# Autodesk Inventor assembly: Frame 1647030135921
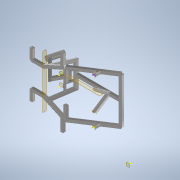
[picture p0: Inventor's stored thumbnail of the model, 180x180]
Saved by Autodesk Inventor 2022.2 (Build 262287000, 287)
## iProperties
_FrameDoc: Frame Assembly
_Version: 25.0.0
Created: 2022-03-11
Part Number: Frame 1647030135921
Document SubType Name: Assembly
Designer: foriw
Mass: 3942.11 g
Surface Area: 4958.76 cm^2
Volume: 504.942 cm^3
Density: 7.80705 g/cm^3
Author: foriw
## Documents named in this file (29)
- C:\Users\foriw\OneDrive\Dokumenter\Inventor\BeerCart - Github - Mekatronik\BeerCart-CAD-Inventor\Workspaces\Workspace\beercart assembly - mekatronik\Frame\Frame 1647030135921.iam
- C:\Users\foriw\OneDrive\Dokumenter\Inventor\BeerCart - Github - Mekatronik\BeerCart-CAD-Inventor\Workspaces\Workspace\beercart assembly - mekatronik\Frame\Skeleton 1647030135922.ipt
- C:\Users\foriw\OneDrive\Dokumenter\Inventor\BeerCart - Github - Mekatronik\BeerCart-CAD-Inventor\Workspaces\Workspace\beercart assembly - mekatronik\Frame\ISO 12633-2 20x20x2 1647030137505.ipt
- C:\Users\foriw\OneDrive\Dokumenter\Inventor\BeerCart - Github - Mekatronik\BeerCart-CAD-Inventor\Workspaces\Workspace\beercart assembly - mekatronik\Frame\ISO 12633-2 20x20x2 1647030138110.ipt
- C:\Users\foriw\OneDrive\Dokumenter\Inventor\BeerCart - Github - Mekatronik\BeerCart-CAD-Inventor\Workspaces\Workspace\beercart assembly - mekatronik\Frame\ISO 12633-2 20x20x2 1647030138225.ipt
- C:\Users\foriw\OneDrive\Dokumenter\Inventor\BeerCart - Github - Mekatronik\BeerCart-CAD-Inventor\Workspaces\Workspace\beercart assembly - mekatronik\Frame\ISO 12633-2 20x20x2 1647030639616.ipt
- C:\Users\foriw\OneDrive\Dokumenter\Inventor\BeerCart - Github - Mekatronik\BeerCart-CAD-Inventor\Workspaces\Workspace\beercart assembly - mekatronik\Frame\ISO 12633-2 20x20x2 1647030639707.ipt
- C:\Users\foriw\OneDrive\Dokumenter\Inventor\BeerCart - Github - Mekatronik\BeerCart-CAD-Inventor\Workspaces\Workspace\beercart assembly - mekatronik\Frame\ISO 1035_2 10x 10 1647602096505.ipt
- C:\Users\foriw\OneDrive\Dokumenter\Inventor\BeerCart - Github - Mekatronik\BeerCart-CAD-Inventor\Workspaces\Workspace\beercart assembly - mekatronik\Frame\ISO 1035_2 10x 10 1647602096566.ipt
- C:\Users\foriw\OneDrive\Dokumenter\Inventor\BeerCart - Github - Mekatronik\BeerCart-CAD-Inventor\Workspaces\Workspace\beercart assembly - mekatronik\Frame\ISO 1035_2 10x 10 1647602096620.ipt
- C:\Users\foriw\OneDrive\Dokumenter\Inventor\BeerCart - Github - Mekatronik\BeerCart-CAD-Inventor\Workspaces\Workspace\beercart assembly - mekatronik\Frame\ISO 12633-2 20x20x2 1647606177319.ipt
- C:\Users\foriw\OneDrive\Dokumenter\Inventor\BeerCart - Github - Mekatronik\BeerCart-CAD-Inventor\Workspaces\Workspace\beercart assembly - mekatronik\Frame\ISO 12633-2 20x20x2 1647606177438.ipt
- C:\Users\foriw\OneDrive\Dokumenter\Inventor\BeerCart - Github - Mekatronik\BeerCart-CAD-Inventor\Workspaces\Workspace\beercart assembly - mekatronik\Frame\FrontWheelFrame.iam
- C:\Users\foriw\OneDrive\Dokumenter\Inventor\BeerCart - Github - Mekatronik\BeerCart-CAD-Inventor\Workspaces\Workspace\beercart assembly - mekatronik\Frame\ISO 12633-2 20x20x2 1648210122933.ipt
- C:\Users\foriw\OneDrive\Dokumenter\Inventor\BeerCart - Github - Mekatronik\BeerCart-CAD-Inventor\Workspaces\Workspace\beercart assembly - mekatronik\Frame\ISO 12633-2 20x20x2 1648210123162.ipt
- C:\Users\foriw\OneDrive\Dokumenter\Inventor\BeerCart - Github - Mekatronik\BeerCart-CAD-Inventor\Workspaces\Workspace\BackWheelMountingPlate.ipt
- C:\Users\foriw\OneDrive\Dokumenter\Inventor\BeerCart - Github - Mekatronik\BeerCart-CAD-Inventor\Workspaces\Workspace\BackWheelMountingPlate_MIR_MIR.ipt
- C:\Users\foriw\OneDrive\Dokumenter\Inventor\BeerCart - Github - Mekatronik\BeerCart-CAD-Inventor\Workspaces\Workspace\beercart assembly - mekatronik\Frame\ISO 1035_2 10x 10 1648211737860.ipt
- C:\Users\foriw\OneDrive\Dokumenter\Inventor\BeerCart - Github - Mekatronik\BeerCart-CAD-Inventor\Workspaces\Workspace\bearing housing front.ipt
- C:\Users\foriw\OneDrive\Dokumenter\Inventor\BeerCart - Github - Mekatronik\BeerCart-CAD-Inventor\Workspaces\Workspace\beercart assembly - mekatronik\Frame\ISO 12633-2 20x20x2 1648404911470.ipt
- C:\Users\foriw\OneDrive\Dokumenter\Inventor\BeerCart - Github - Mekatronik\BeerCart-CAD-Inventor\Workspaces\Workspace\beercart assembly - mekatronik\Frame\ISO 12633-2 20x20x2 1648404911558.ipt
- C:\Users\foriw\OneDrive\Dokumenter\Inventor\BeerCart - Github - Mekatronik\BeerCart-CAD-Inventor\Workspaces\Workspace\beercart assembly - mekatronik\Frame\ISO 12633-2 20x20x2 1648404911659.ipt
- C:\Users\foriw\OneDrive\Dokumenter\Inventor\BeerCart - Github - Mekatronik\BeerCart-CAD-Inventor\Workspaces\Workspace\beercart assembly - mekatronik\Frame\ISO 12633-2 20x20x2 1648404911754.ipt
- C:\Users\foriw\OneDrive\Dokumenter\Inventor\BeerCart - Github - Mekatronik\BeerCart-CAD-Inventor\Workspaces\Workspace\beercart assembly - mekatronik\Frame\ISO 12633-2 20x20x2 1648404911848.ipt
- C:\Users\foriw\OneDrive\Dokumenter\Inventor\BeerCart - Github - Mekatronik\BeerCart-CAD-Inventor\Workspaces\Workspace\beercart assembly - mekatronik\Frame\ISO 12633-2 20x20x2 1648404911940.ipt
- C:\Users\foriw\OneDrive\Dokumenter\Inventor\BeerCart - Github - Mekatronik\BeerCart-CAD-Inventor\Workspaces\Workspace\beercart assembly - mekatronik\Frame\ISO 12633-2 20x20x2 1648573909221.ipt
- C:\Users\foriw\OneDrive\Dokumenter\Inventor\BeerCart - Github - Mekatronik\BeerCart-CAD-Inventor\Workspaces\Workspace\beercart assembly - mekatronik\Frame\ISO 12633-2 20x20x2 1648573975084.ipt
- C:\Users\foriw\OneDrive\Dokumenter\Inventor\BeerCart - Github - Mekatronik\BeerCart-CAD-Inventor\Workspaces\Workspace\BackWheelMountingPlate_MIR3.ipt
- C:\Users\foriw\OneDrive\Dokumenter\Inventor\BeerCart - Github - Mekatronik\BeerCart-CAD-Inventor\Workspaces\Workspace\beercart assembly - mekatronik\Frame\ISO 12633-2 20x20x2 1648580035059.ipt
## Components (31 placed, 19 different names)
1. bearing housing front:1 — Rotational:1
2. Reference Skeleton
3. ISO 12633-2 20x20x2 - 310:2
4. ISO 12633-2 20x20x2 - 290:1
5. ISO 12633-2 20x20x2 - 185.38:3
6. ISO 12633-2 20x20x2 - 166.84:1
7. ISO 12633-2 20x20x2 - 166.84:2
8. ISO 1035/2 10x 10 - 58.59:1
9. ISO 1035/2 10x 10 - 43.59:1
10. ISO 1035/2 10x 10 - 43.59:2
11. ISO 12633-2 20x20x2 - 164,49:1 — Mate:1, Mate:3
12. ISO 12633-2 20x20x2 - 164,49:2 — Mate:2, Mate:4, Mate:5
13. BackWheelMountingPlate:1 — Flush:6, Rotational:2
14. FrontWheelFrame:1 [sub-assembly] — Rotational:1
15. ISO 12633-2 20x20x2 - 87:1
16. ISO 12633-2 20x20x2 - 87:2
17. BackWheelMountingPlate_MIR_MIR:1
18. ISO 1035/2 10x 10 - 58.59:1
19. ISO 12633-2 20x20x2 - 80:1
20. ISO 12633-2 20x20x2 - 80:2
21. ISO 12633-2 20x20x2 - 80:3
22. ISO 12633-2 20x20x2 - 70:1
23. ISO 12633-2 20x20x2 - 80:4
24. ISO 12633-2 20x20x2 - 70:2
25. ISO 12633-2 20x20x2 - 274,59:1
26. ISO 12633-2 20x20x2 - 44,58:1 — Flush:6, Rotational:2
27. BackWheelMountingPlate_MIR3:1 — Flush:8, Rotational:4
28. ISO 12633-2 20x20x2 - 274,59:3
29. ISO 12633-2 20x20x2 - 44,58:3 — Flush:8, Rotational:4
30. ISO 12633-2 20x20x2 - 115,85:1
31. ISO 12633-2 20x20x2 - 115,85:2
## Relationships (12: Mate 6, Flush 3, RevoluteJoint 3)
- Mate:1: ISO 12633-2 20x20x2 - 164,49:1
- Mate:2: ISO 12633-2 20x20x2 - 164,49:2
- Mate:3: ISO 12633-2 20x20x2 - 164,49:1
- Mate:4: ISO 12633-2 20x20x2 - 164,49:2
- Mate:5: ISO 12633-2 20x20x2 - 164,49:2
- [Mate]: bearing housing front:1 ↔ ISO 1035/2 10x 10 - 58.59:1
- [Flush] (1 mm): bearing housing front:1 ↔ ISO 1035/2 10x 10 - 58.59:1
- Rotational:1 [RevoluteJoint] (4 mm): bearing housing front:1 ↔ FrontWheelFrame:1
- Flush:6: BackWheelMountingPlate:1 ↔ ISO 12633-2 20x20x2 - 44,58:1
- Rotational:2 [RevoluteJoint]: BackWheelMountingPlate:1 ↔ ISO 12633-2 20x20x2 - 44,58:1
- Flush:8: BackWheelMountingPlate_MIR3:1 ↔ ISO 12633-2 20x20x2 - 44,58:3
- Rotational:4 [RevoluteJoint]: BackWheelMountingPlate_MIR3:1 ↔ ISO 12633-2 20x20x2 - 44,58:3
## Named parameters: d22_d2 = 0 mm, d23_d3 = 1 mm
